# Autodesk Inventor assembly: I6ABreakout
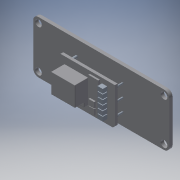
[picture p0: Inventor's stored thumbnail of the model, 180x180]
Saved by Autodesk Inventor 2018 (Build 220112000, 112)
## iProperties
Created: 2017-11-11
Part Number: I6ABreakout
Document SubType Name: Assembly
Designer: lsullivan
Author: lsullivan
## Documents named in this file (3)
- C:\Users\lsullivan\Workspace\I6ABreakout\I6ABreakout.iam
- C:\Users\lsullivan\Workspace\I6ABreakout\i6a_standard_asm.ipt
- C:\Users\lsullivan\Workspace\I6ABreakout\I6ABreakout.ipt
## Components (2 placed, 2 different names)
1. I6ABreakout:2 — Mate:1, Mate:2, Mate:3, Mate:4
2. i6a_standard_asm:1 — Mate:1, Mate:2, Mate:3, Mate:4
## Relationships (4: Mate 4)
- Mate:1: I6ABreakout:2 ↔ i6a_standard_asm:1
- Mate:2 (-8.8138 mm): I6ABreakout:2 ↔ i6a_standard_asm:1
- Mate:3 (-15.3416 mm): I6ABreakout:2 ↔ i6a_standard_asm:1
- Mate:4 (-27.8892 mm): I6ABreakout:2 ↔ i6a_standard_asm:1
